# Autodesk Inventor assembly: Test slider
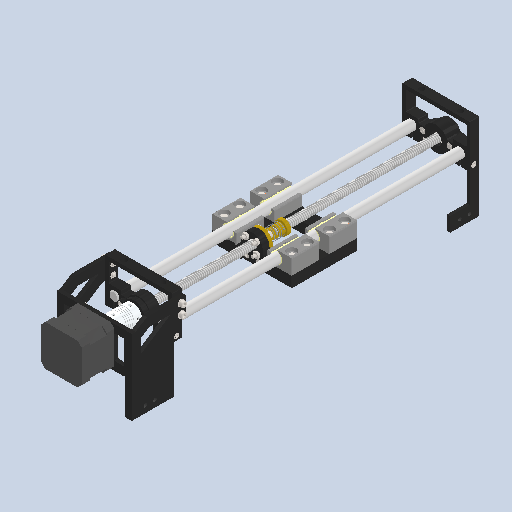
[picture p0: Inventor's stored thumbnail of the model, 512x512]
Saved by Autodesk Inventor 2023 (Build 270158000, 158)
## iProperties
Created: 2018-08-24
Part Number: Test slider
Description: STEP AP214
Document SubType Name: Assembly
Designer: Ayoub
Sending System: SolidWorks 2017
Preprocessor: SwSTEP 2.0
Title: Test slider.STEP
Revision Number: ANY
## Documents named in this file (24)
- C:\Users\Ayoub\Documents\GitHub\zonnepaneel-concept\Parts\Test slider\Test slider.iam
- C:\Users\Ayoub\Documents\GitHub\zonnepaneel-concept\Parts\Nema17 Stepper motor.ipt
- C:\Users\Ayoub\Documents\GitHub\zonnepaneel-concept\Parts\Flexible coupling D20 d5.ipt
- C:\Users\Ayoub\Documents\GitHub\zonnepaneel-concept\Parts\radial ball bearing_68_skf_SKF - 626 - 8,SI,NC,8_68.ipt
- C:\Users\Ayoub\Documents\GitHub\zonnepaneel-concept\Parts\hex thin nut chamfered gradeab_din_Hexagon Thin Nut ISO 4035 - M6 - N.ipt
- C:\Users\Ayoub\Documents\GitHub\zonnepaneel-concept\Parts\radial ball bearing_68_skf_SKF - 618-8 - 12,SI,NC,12_68.ipt
- C:\Users\Ayoub\Documents\GitHub\zonnepaneel-concept\Parts\T8 Antibacklash nut.iam
- C:\Users\Ayoub\Documents\GitHub\zonnepaneel-concept\Parts\WJ200UM_01_10_2.ipt
- C:\Users\Ayoub\Documents\GitHub\zonnepaneel-concept\Parts\Test slider support 1.ipt
- C:\Users\Ayoub\Documents\GitHub\zonnepaneel-concept\Parts\Test slider carriage small_double.ipt
- C:\Users\Ayoub\Documents\GitHub\zonnepaneel-concept\Parts\socket head cap screw_din_DIN 912 M6 x 16 --- 16N.ipt
- C:\Users\Ayoub\Documents\GitHub\zonnepaneel-concept\Parts\Test slider nut bracket.ipt
- C:\Users\Ayoub\Documents\GitHub\zonnepaneel-concept\Parts\socket head cap screw_din_DIN 912 M3 x 16 --- 16N.ipt
- C:\Users\Ayoub\Documents\GitHub\zonnepaneel-concept\Parts\hex nut style 1 gradeab_din_Hexagon Nut ISO 4032 - M3 - D - N.ipt
- C:\Users\Ayoub\Documents\GitHub\zonnepaneel-concept\Parts\socket head cap screw_din_DIN 912 M3 x 10 --- 10N.ipt
- C:\Users\Ayoub\Documents\GitHub\zonnepaneel-concept\Parts\Test slider support 1 cover.ipt
- C:\Users\Ayoub\Documents\GitHub\zonnepaneel-concept\Parts\socket head cap screw_din_DIN 912 M3 x 12 --- 12N.ipt
- C:\Users\Ayoub\Documents\GitHub\zonnepaneel-concept\Parts\Test slider support 2.ipt
- C:\Users\Ayoub\Documents\GitHub\zonnepaneel-concept\Parts\Test slider support 2 cover.ipt
- C:\Users\Ayoub\Documents\GitHub\zonnepaneel-concept\Parts\Test slider stepper mount.ipt
- C:\Users\Ayoub\Documents\GitHub\zonnepaneel-concept\Parts\plain washer grade a_din_Washer DIN 125 - A 3.2.ipt
- C:\Users\Ayoub\Documents\GitHub\zonnepaneel-concept\Parts\Staaf.ipt
- C:\Users\Ayoub\Documents\GitHub\zonnepaneel-concept\Parts\Part2.ipt
- C:\Users\Ayoub\Documents\GitHub\zonnepaneel-concept\Parts\leadscrew part2.ipt
## Components (77 placed, 76 different names)
1. Nema17 Stepper motor_1
2. Flexible coupling D20 d5_2
3. radial ball bearing_68_skf_SKF - 626 - 8,SI,NC,8_68_4 — Insert:33
4. hex thin nut chamfered gradeab_din_Hexagon Thin Nut ISO 4035 - M6 - N_5
5. radial ball bearing_68_skf_SKF - 618-8 - 12,SI,NC,12_68_6 — Insert:34
6. T8 Antibacklash nut_8 [sub-assembly] — Mate:2, Mate:3, Insert:1, Insert:2, Insert:3, Insert:4
7. WJ200UM_01_10_2_9 — Insert:17, Mate:20
8. Test slider support 1_11 — Insert:34, Mate:22, Insert:39, Insert:40, Insert:43
9. WJ200UM_01_10_2_12 — Insert:23, Insert:30
10. Test slider carriage small_double_13 — Mate:10, Mate:11, Insert:9, Insert:10, Insert:11, Insert:12, Insert:13, Insert:14, Insert:15, Insert:16
11. socket head cap screw_din_DIN 912 M6 x 16 --- 16N_14 — Insert:14, Insert:17
12. socket head cap screw_din_DIN 912 M6 x 16 --- 16N_15 — Insert:13
13. socket head cap screw_din_DIN 912 M6 x 16 --- 16N_16 — Insert:9, Insert:23
14. socket head cap screw_din_DIN 912 M6 x 16 --- 16N_17 — Insert:10, Insert:30
15. Test slider nut bracket_18 — Mate:2, Mate:3, Mate:6, Mate:7, Mate:8, Mate:9, Insert:5, Insert:6, Mate:21
16. socket head cap screw_din_DIN 912 M3 x 16 --- 16N_19 — Insert:4
17. socket head cap screw_din_DIN 912 M3 x 16 --- 16N_20 — Insert:3
18. socket head cap screw_din_DIN 912 M3 x 16 --- 16N_21 — Insert:1
19. socket head cap screw_din_DIN 912 M3 x 16 --- 16N_22 — Insert:2
20. hex nut style 1 gradeab_din_Hexagon Nut ISO 4032 - M3 - D - N_23 — Mate:7
21. hex nut style 1 gradeab_din_Hexagon Nut ISO 4032 - M3 - D - N_24 — Mate:9
22. hex nut style 1 gradeab_din_Hexagon Nut ISO 4032 - M3 - D - N_25 — Mate:6
23. hex nut style 1 gradeab_din_Hexagon Nut ISO 4032 - M3 - D - N_26 — Mate:8
24. socket head cap screw_din_DIN 912 M3 x 10 --- 10N_27 — Insert:6, Insert:7
25. socket head cap screw_din_DIN 912 M3 x 10 --- 10N_28 — Insert:5, Insert:8
26. hex nut style 1 gradeab_din_Hexagon Nut ISO 4032 - M3 - D - N_29 — Insert:42
27. socket head cap screw_din_DIN 912 M3 x 16 --- 16N_30 — Insert:39, Insert:42
28. socket head cap screw_din_DIN 912 M3 x 16 --- 16N_31 — Insert:40, Insert:41
29. hex nut style 1 gradeab_din_Hexagon Nut ISO 4032 - M3 - D - N_32 — Insert:41
30. Test slider support 1 cover_33 — Mate:22, Insert:35, Insert:36
31. socket head cap screw_din_DIN 912 M3 x 12 --- 12N_34 — Insert:35, Insert:37
32. socket head cap screw_din_DIN 912 M3 x 12 --- 12N_35 — Insert:36, Insert:38
33. hex nut style 1 gradeab_din_Hexagon Nut ISO 4032 - M3 - D - N_36 — Insert:38
34. hex nut style 1 gradeab_din_Hexagon Nut ISO 4032 - M3 - D - N_37 — Insert:37
35. Test slider support 2_38 — Insert:20, Insert:27, Insert:31, Insert:32
36. Test slider support 2 cover_39
37. Test slider stepper mount_40 — Insert:20, Mate:18, Mate:19, Insert:27
38. plain washer grade a_din_Washer DIN 125 - A 3.2_41
39. plain washer grade a_din_Washer DIN 125 - A 3.2_42
40. plain washer grade a_din_Washer DIN 125 - A 3.2_43
41. plain washer grade a_din_Washer DIN 125 - A 3.2_44
42. socket head cap screw_din_DIN 912 M3 x 10 --- 10N_45
43. socket head cap screw_din_DIN 912 M3 x 10 --- 10N_46
44. socket head cap screw_din_DIN 912 M3 x 10 --- 10N_47
45. socket head cap screw_din_DIN 912 M3 x 10 --- 10N_48
46. plain washer grade a_din_Washer DIN 125 - A 3.2_49
47. plain washer grade a_din_Washer DIN 125 - A 3.2_50
48. socket head cap screw_din_DIN 912 M3 x 10 --- 10N_51
49. socket head cap screw_din_DIN 912 M3 x 10 --- 10N_52
50. hex nut style 1 gradeab_din_Hexagon Nut ISO 4032 - M3 - D - N_53
51. hex nut style 1 gradeab_din_Hexagon Nut ISO 4032 - M3 - D - N_54
52. hex nut style 1 gradeab_din_Hexagon Nut ISO 4032 - M3 - D - N_55
53. hex nut style 1 gradeab_din_Hexagon Nut ISO 4032 - M3 - D - N_56
54. hex nut style 1 gradeab_din_Hexagon Nut ISO 4032 - M3 - D - N_57
55. hex nut style 1 gradeab_din_Hexagon Nut ISO 4032 - M3 - D - N_58
56. socket head cap screw_din_DIN 912 M3 x 16 --- 16N_59
57. socket head cap screw_din_DIN 912 M3 x 16 --- 16N_60
58. socket head cap screw_din_DIN 912 M3 x 12 --- 12N_61
59. socket head cap screw_din_DIN 912 M3 x 12 --- 12N_62
60. plain washer grade a_din_Washer DIN 125 - A 3.2_63 — Mate:18, Insert:21
61. plain washer grade a_din_Washer DIN 125 - A 3.2_64 — Mate:19, Insert:22
62. socket head cap screw_din_DIN 912 M3 x 10 --- 10N_65 — Insert:21
63. socket head cap screw_din_DIN 912 M3 x 10 --- 10N_66 — Insert:22
64. hex nut style 1 gradeab_din_Hexagon Nut ISO 4032 - M3 - D - N_67
65. hex nut style 1 gradeab_din_Hexagon Nut ISO 4032 - M3 - D - N_68
66. socket head cap screw_din_DIN 912 M6 x 16 --- 16N_69 — Insert:16, Insert:28
67. socket head cap screw_din_DIN 912 M6 x 16 --- 16N_70 — Insert:15, Insert:24
68. socket head cap screw_din_DIN 912 M6 x 16 --- 16N_71 — Insert:11, Insert:29
69. socket head cap screw_din_DIN 912 M6 x 16 --- 16N_72 — Insert:12, Insert:25
70. WJ200UM_01_10_2_73 — Insert:25, Insert:29
71. WJ200UM_01_10_2_74 — Insert:24, Insert:28
72. hex nut style 1 gradeab_din_Hexagon Nut ISO 4032 - M3 - D - N_75 — Mate:10, Insert:7
73. hex nut style 1 gradeab_din_Hexagon Nut ISO 4032 - M3 - D - N_76 — Mate:11, Insert:8
74. Staaf:1 — Insert:32, Mate:20, Insert:43
75. Staaf:2 — Insert:31
76. Part2:1
77. leadscrew part2:1 — Insert:33, Mate:21
## Relationships (53: Insert 40, Mate 13)
- Mate:2: T8 Antibacklash nut_8 ↔ Test slider nut bracket_18
- Mate:3: T8 Antibacklash nut_8 ↔ Test slider nut bracket_18
- Insert:1: T8 Antibacklash nut_8 ↔ socket head cap screw_din_DIN 912 M3 x 16 --- 16N_21
- Insert:2: T8 Antibacklash nut_8 ↔ socket head cap screw_din_DIN 912 M3 x 16 --- 16N_22
- Mate:6: Test slider nut bracket_18 ↔ hex nut style 1 gradeab_din_Hexagon Nut ISO 4032 - M3 - D - N_25
- Mate:7: Test slider nut bracket_18 ↔ hex nut style 1 gradeab_din_Hexagon Nut ISO 4032 - M3 - D - N_23
- Mate:8: Test slider nut bracket_18 ↔ hex nut style 1 gradeab_din_Hexagon Nut ISO 4032 - M3 - D - N_26
- Insert:3: T8 Antibacklash nut_8 ↔ socket head cap screw_din_DIN 912 M3 x 16 --- 16N_20
- Insert:4: T8 Antibacklash nut_8 ↔ socket head cap screw_din_DIN 912 M3 x 16 --- 16N_19
- Mate:9: Test slider nut bracket_18 ↔ hex nut style 1 gradeab_din_Hexagon Nut ISO 4032 - M3 - D - N_24
- Insert:5: Test slider nut bracket_18 ↔ socket head cap screw_din_DIN 912 M3 x 10 --- 10N_28
- Insert:6: Test slider nut bracket_18 ↔ socket head cap screw_din_DIN 912 M3 x 10 --- 10N_27
- Mate:10: Test slider carriage small_double_13 ↔ hex nut style 1 gradeab_din_Hexagon Nut ISO 4032 - M3 - D - N_75
- Mate:11: Test slider carriage small_double_13 ↔ hex nut style 1 gradeab_din_Hexagon Nut ISO 4032 - M3 - D - N_76
- Insert:7: socket head cap screw_din_DIN 912 M3 x 10 --- 10N_27 ↔ hex nut style 1 gradeab_din_Hexagon Nut ISO 4032 - M3 - D - N_75
- Insert:8: socket head cap screw_din_DIN 912 M3 x 10 --- 10N_28 ↔ hex nut style 1 gradeab_din_Hexagon Nut ISO 4032 - M3 - D - N_76
- Insert:9: Test slider carriage small_double_13 ↔ socket head cap screw_din_DIN 912 M6 x 16 --- 16N_16
- Insert:10: Test slider carriage small_double_13 ↔ socket head cap screw_din_DIN 912 M6 x 16 --- 16N_17
- Insert:11: Test slider carriage small_double_13 ↔ socket head cap screw_din_DIN 912 M6 x 16 --- 16N_71
- Insert:12: Test slider carriage small_double_13 ↔ socket head cap screw_din_DIN 912 M6 x 16 --- 16N_72
- Insert:13: Test slider carriage small_double_13 ↔ socket head cap screw_din_DIN 912 M6 x 16 --- 16N_15
- Insert:14: Test slider carriage small_double_13 ↔ socket head cap screw_din_DIN 912 M6 x 16 --- 16N_14
- Insert:15: Test slider carriage small_double_13 ↔ socket head cap screw_din_DIN 912 M6 x 16 --- 16N_70
- Insert:16: Test slider carriage small_double_13 ↔ socket head cap screw_din_DIN 912 M6 x 16 --- 16N_69
- Insert:17 (-2.5 mm): WJ200UM_01_10_2_9 ↔ socket head cap screw_din_DIN 912 M6 x 16 --- 16N_14
- Insert:20: Test slider support 2_38 ↔ Test slider stepper mount_40
- Mate:18: Test slider stepper mount_40 ↔ plain washer grade a_din_Washer DIN 125 - A 3.2_63
- Insert:21: plain washer grade a_din_Washer DIN 125 - A 3.2_63 ↔ socket head cap screw_din_DIN 912 M3 x 10 --- 10N_65
- Mate:19: Test slider stepper mount_40 ↔ plain washer grade a_din_Washer DIN 125 - A 3.2_64
- Insert:22: plain washer grade a_din_Washer DIN 125 - A 3.2_64 ↔ socket head cap screw_din_DIN 912 M3 x 10 --- 10N_66
- Insert:23: WJ200UM_01_10_2_12 ↔ socket head cap screw_din_DIN 912 M6 x 16 --- 16N_16
- Insert:24: socket head cap screw_din_DIN 912 M6 x 16 --- 16N_70 ↔ WJ200UM_01_10_2_74
- Insert:25: socket head cap screw_din_DIN 912 M6 x 16 --- 16N_72 ↔ WJ200UM_01_10_2_73
- Insert:27: Test slider support 2_38 ↔ Test slider stepper mount_40
- Insert:28: socket head cap screw_din_DIN 912 M6 x 16 --- 16N_69 ↔ WJ200UM_01_10_2_74
- Insert:29: socket head cap screw_din_DIN 912 M6 x 16 --- 16N_71 ↔ WJ200UM_01_10_2_73
- Insert:30: WJ200UM_01_10_2_12 ↔ socket head cap screw_din_DIN 912 M6 x 16 --- 16N_17
- Insert:31: Test slider support 2_38 ↔ Staaf:2
- Insert:32: Test slider support 2_38 ↔ Staaf:1
- Mate:20: WJ200UM_01_10_2_9 ↔ Staaf:1
- Insert:33: radial ball bearing_68_skf_SKF - 626 - 8,SI,NC,8_68_4 ↔ leadscrew part2:1
- Mate:21: Test slider nut bracket_18 ↔ leadscrew part2:1
- Insert:34: radial ball bearing_68_skf_SKF - 618-8 - 12,SI,NC,12_68_6 ↔ Test slider support 1_11
- Mate:22: Test slider support 1_11 ↔ Test slider support 1 cover_33
- Insert:35: Test slider support 1 cover_33 ↔ socket head cap screw_din_DIN 912 M3 x 12 --- 12N_34
- Insert:36: Test slider support 1 cover_33 ↔ socket head cap screw_din_DIN 912 M3 x 12 --- 12N_35
- Insert:37: socket head cap screw_din_DIN 912 M3 x 12 --- 12N_34 ↔ hex nut style 1 gradeab_din_Hexagon Nut ISO 4032 - M3 - D - N_37
- Insert:38: socket head cap screw_din_DIN 912 M3 x 12 --- 12N_35 ↔ hex nut style 1 gradeab_din_Hexagon Nut ISO 4032 - M3 - D - N_36
- Insert:39: Test slider support 1_11 ↔ socket head cap screw_din_DIN 912 M3 x 16 --- 16N_30
- Insert:40: Test slider support 1_11 ↔ socket head cap screw_din_DIN 912 M3 x 16 --- 16N_31
- Insert:41: socket head cap screw_din_DIN 912 M3 x 16 --- 16N_31 ↔ hex nut style 1 gradeab_din_Hexagon Nut ISO 4032 - M3 - D - N_32
- Insert:42: hex nut style 1 gradeab_din_Hexagon Nut ISO 4032 - M3 - D - N_29 ↔ socket head cap screw_din_DIN 912 M3 x 16 --- 16N_30
- Insert:43: Test slider support 1_11 ↔ Staaf:1
